# Autodesk Inventor assembly: Hand_tyokudou
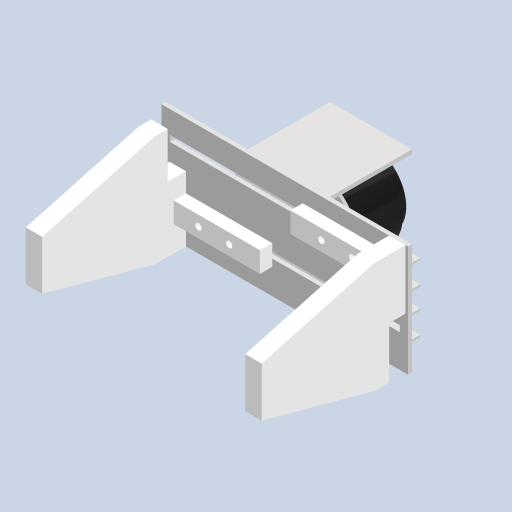
[picture p0: Inventor's stored thumbnail of the model, 512x512]
Saved by Autodesk Inventor 2023 (Build 270158000, 158)
## iProperties
Created: 2024-11-27
Part Number: Hand_tyokudou
Document SubType Name: Assembly
Designer: kiyo
Author: kiyo
## Documents named in this file (8)
- D:\GitHub\inventor\syu-si\OfficeRobot\Manipulator\Hand_tyokudou.iam
- D:\GitHub\inventor\syu-si\OfficeRobot\ReadyMade\Steadywin\GIM3505-8_with-driver.ipt
- D:\GitHub\inventor\syu-si\OfficeRobot\Manipulator\rackgear.ipt
- D:\GitHub\inventor\syu-si\OfficeRobot\Manipulator\motor-fixing.ipt
- D:\GitHub\inventor\syu-si\OfficeRobot\Manipulator\hand-box.ipt
- D:\GitHub\inventor\syu-si\OfficeRobot\Manipulator\left-nail.ipt
- D:\GitHub\inventor\syu-si\OfficeRobot\Manipulator\right-nail.ipt
- D:\GitHub\inventor\syu-si\OfficeRobot\Manipulator\hand-gear.ipt
## Components (8 placed, 7 different names)
1. GIM3505-8_with-driver:1 — 角度:3, 挿入:2, 挿入:3
2. left-nail:1
3. right-nail:1
4. hand-box:1
5. rackgear:1 — 角度:2
6. rackgear:2 — 角度:1
7. hand-gear
8. motor-fixing:1 — 挿入:2, 挿入:3
## Relationships (17: Insert 9, Mate 5, Angle 3)
- 角度:1 [Angle] (0 deg): rackgear:2
- 角度:2 [Angle] (180 deg): rackgear:1
- [Mate]: hand-box:1 ↔ rackgear:2
- [Mate]: hand-box:1 ↔ rackgear:1
- [Insert]: GIM3505-8_with-driver:1 ↔ hand-gear
- [Mate] (0.05 mm): hand-box:1 ↔ rackgear:2
- [Mate] (0.05 mm): hand-box:1 ↔ rackgear:1
- 角度:3 [Angle] (0 deg): GIM3505-8_with-driver:1
- 挿入:2 [Insert]: GIM3505-8_with-driver:1 ↔ motor-fixing:1
- 挿入:3 [Insert]: GIM3505-8_with-driver:1 ↔ motor-fixing:1
- [Mate] (1 mm): rackgear:2 ↔ hand-gear
- [Insert]: hand-box:1 ↔ motor-fixing:1
- [Insert]: hand-box:1 ↔ motor-fixing:1
- [Insert] (2 mm): left-nail:1 ↔ rackgear:2
- [Insert] (2 mm): left-nail:1 ↔ rackgear:2
- [Insert] (2 mm): right-nail:1 ↔ rackgear:1
- [Insert] (2 mm): right-nail:1 ↔ rackgear:1
